# Autodesk Inventor assembly: Piston
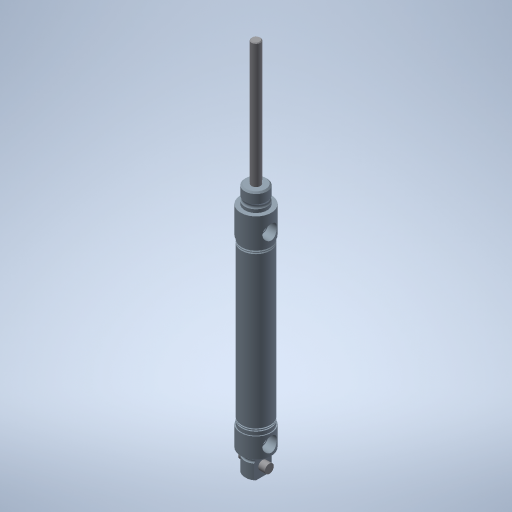
[picture p0: Inventor's stored thumbnail of the model, 512x512]
Saved by Autodesk Inventor 2023 (Build 270158000, 158)
## iProperties
Company: TraceParts S.A.
Created: 2022-06-09
Part Number: Piston
Checked By: TraceParts S.A.
Catalog Web Link: www.traceparts.com
Document SubType Name: Assembly
Designer: TraceParts
DESIGN: NITRA pneumatic cylinder, non-repairable, 3/4in bore, 1/4in rod diameter, 3in stroke, double acting, rear pivot mount.
Part_Number_EShop_URL: http://www.adcpn.com/pn/A12030DP
SUPPLIER_PART_NUMBER: A12030DP
SUPPLIER_NAME: AutomationDirect
Author: TraceParts
## Documents named in this file (4)
- C:\Users\Gabriel - T3 CAD\Documents\GitHub\t3-CAD\T3-CAD\Stock\Pneumatics\Piston.iam
- C:\Users\Gabriel - T3 CAD\Documents\133298157-9-a12030dp\a12030dp_01.ipt
- C:\Users\Gabriel - T3 CAD\Documents\133298157-9-a12030dp\a12030dp_02.ipt
- C:\Users\Gabriel - T3 CAD\Documents\133298157-9-a12030dp\a12030dp_03.ipt
## Components (3 placed, 3 different names)
1. a12030dp_01:1 — Mate:1, Mate:2, Rigid:1
2. a12030dp_02:1 — Mate:1, Mate:2, Rigid:1
3. a12030dp_03:1
## Relationships (3: Mate 2, WeldJoint 1)
- Mate:1: a12030dp_01:1 ↔ a12030dp_02:1
- Mate:2: a12030dp_01:1 ↔ a12030dp_02:1
- Rigid:1 [WeldJoint]: a12030dp_01:1 ↔ a12030dp_02:1
